# Autodesk Inventor assembly: PLA_SetColor_8_穴付き
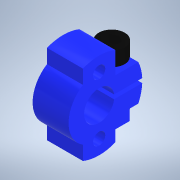
[picture p0: Inventor's stored thumbnail of the model, 180x180]
Saved by Autodesk Inventor 2022.3 (Build 263350000, 350)
## iProperties
Created: 2020-12-13
Part Number: PLA_SetColor_8_穴付き
Document SubType Name: Assembly
Designer: Hagihara Yuya
Author: Hagihara Yuya
## Documents named in this file (4)
- C:\Users\YusukeKunita\Documents\GrabCAD\NHK2022\BasicParts\SetCollar\PLA_SetCollar_d8\PLA_SetColor_d8_穴付き.iam
- C:\Users\YusukeKunita\Documents\GrabCAD\NHK2022\BasicParts\SetCollar\PLA_SetCollar_d8\PLA_SetColor_d8_穴付き.ipt
- C:\Users\YusukeKunita\Documents\GrabCAD\NHK2022\BasicParts\SetCollar\PLA_SetCollar_d8\Bolt_M4_15_for_SetCollar_d8.ipt
- C:\Users\YusukeKunita\Documents\GrabCAD\NHK2022\BasicParts\SetCollar\PLA_SetCollar_d8\Nut_M4_for_SetCollar.ipt
## Components (3 placed, 3 different names)
1. PLA_SetColor_d8_穴付き:1 — 回転:1, 回転:2
2. Bolt_M4_15_for_SetCollar_d8:1 — 回転:1
3. Nut_M4_for_SetCollar:1 — 回転:2
## Relationships (2: RevoluteJoint 2)
- 回転:1 [RevoluteJoint]: PLA_SetColor_d8_穴付き:1 ↔ Bolt_M4_15_for_SetCollar_d8:1
- 回転:2 [RevoluteJoint]: PLA_SetColor_d8_穴付き:1 ↔ Nut_M4_for_SetCollar:1
